# Autodesk Inventor assembly: Assembly_carcasa
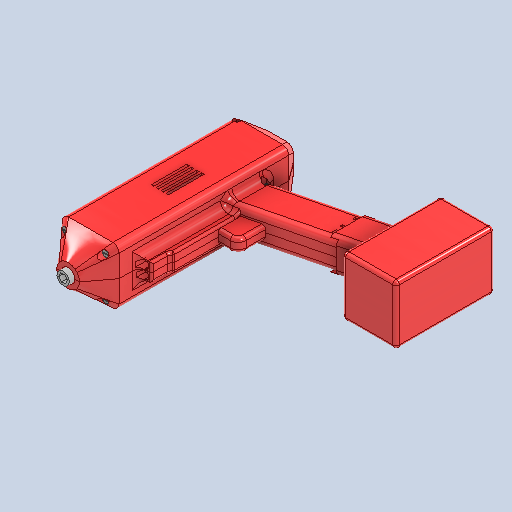
[picture p0: Inventor's stored thumbnail of the model, 512x512]
Saved by Autodesk Inventor 2025.2 (Build 292293000, 293)
## iProperties
Created: 2024-04-15
Part Number: Assembly_carcasa
Document SubType Name: Assembly
Designer: mirun
Author: mirun
## Documents named in this file (17)
- C:\Users\mirewn\Documents\GitHub\Electric-Screwdriver\Assembly.iam
- C:\Users\mirewn\Documents\Inventor\Content Center Files\R2025\en-US\DIN 439-2\DIN 439 - M3 x 0.5.ipt
- C:\Users\mirewn\Documents\Inventor\Content Center Files\R2025\en-US\DIN 934\DIN 934 - M3 x 0.5.ipt
- C:\Users\mirewn\Documents\Inventor\Content Center Files\R2025\en-US\DIN 963\DIN 963 - M3 x 16.ipt
- C:\Users\mirewn\Documents\Inventor\Content Center Files\R2025\en-US\DIN 912\DIN 912 - M3 x 0.5 x 12 x 10.75.ipt
- C:\Users\mirewn\Documents\Inventor\Content Center Files\R2025\en-US\DIN 912\DIN 912 - M3 x 0.5 x 30 x 18.ipt
- C:\Users\mirewn\Documents\Inventor\Content Center Files\R2025\en-US\DIN 912\DIN 912 - M3 x 0.5 x 20 x 18.75.ipt
- C:\Users\mirewn\Documents\Inventor\Content Center Files\R2025\en-US\DIN 912\DIN 912 - M3 x 0.5 x 16 x 14.75.ipt
- C:\Users\mirewn\Documents\GitHub\Electric-Screwdriver\battery_pack_lid.ipt
- C:\Users\mirewn\Documents\GitHub\Electric-Screwdriver\case_R.ipt
- C:\Users\mirewn\Documents\GitHub\Electric-Screwdriver\button.ipt
- C:\Users\mirewn\Documents\GitHub\Electric-Screwdriver\bit_adaptor.ipt
- C:\Users\mirewn\Documents\GitHub\Electric-Screwdriver\bit_adaptor_lid.ipt
- C:\Users\mirewn\Documents\GitHub\Electric-Screwdriver\case_L.ipt
- C:\Users\mirewn\Documents\GitHub\Electric-Screwdriver\GearBox\Assembly.iam
- C:\Users\mirewn\Documents\GitHub\Electric-Screwdriver\battery.ipt
- C:\Users\mirewn\Documents\GitHub\Electric-Screwdriver\battery_pack.ipt
## Components (32 placed, 16 different names)
1. case_R:1 — Mate:3, Mate:4, Flush:2, Mate:12, Mate:13, Flush:3, Flush:4, Mate:30, Mate:31, Mate:32, Mate:36, Mate:37, Mate:45, Mate:46, Mate:49, Mate:50, Mate:52, Mate:55, Insert:13, Insert:14
2. button:1 — Mate:3, Mate:4, Flush:2, Mate:45, Mate:46
3. bit_adaptor:1 — Mate:8, Mate:9, Mate:10, Mate:12, Mate:33
4. bit_adaptor_lid:1 — Mate:8, Mate:9, Mate:10
5. case_L:1 — Mate:13, Flush:3, Flush:4, Mate:35, Mate:47, Mate:48, Mate:51, Mate:53, Mate:54, Insert:15
6. DIN 934 - replaced by DIN EN 24032/28673/28674 M3:1 — Mate:53, Mate:54
7. DIN 934 - replaced by DIN EN 24032/28673/28674 M3:2 — Mate:51
8. DIN 934 - replaced by DIN EN 24032/28673/28674 M3:3 — Mate:52, Mate:55
9. Assembly:1 [sub-assembly] — Mate:30, Mate:31, Mate:32, Mate:33, Insert:1, Insert:2, Insert:3, Insert:4, Insert:5, Insert:6, Insert:7, Insert:8, Insert:9, Insert:10, Insert:11, Insert:12
10. battery:1 — Flush:5, Flush:6, Mate:34, Mate:42, Mate:43, Mate:44
11. battery:2 — Flush:5, Flush:6, Mate:34
12. battery_pack:1 — Mate:35, Mate:36, Mate:37, Mate:39, Mate:40, Mate:41, Mate:42, Mate:43, Mate:44
13. battery_pack_lid:1 — Mate:39, Mate:40, Mate:41
14. DIN 963 - replaced by DIN EN ISO 2009 M3 x 16:1 — Mate:47
15. DIN 963 - replaced by DIN EN ISO 2009 M3 x 16:2 — Mate:48
16. DIN 963 - replaced by DIN EN ISO 2009 M3 x 16:3 — Mate:49
17. DIN 963 - replaced by DIN EN ISO 2009 M3 x 16:4 — Mate:50
18. DIN 439-2 - replaced by DIN EN 24035/28675 M3:1 — Insert:1
19. DIN 439-2 - replaced by DIN EN 24035/28675 M3:2 — Insert:2
20. DIN 439-2 - replaced by DIN EN 24035/28675 M3:3 — Insert:3
21. DIN 439-2 - replaced by DIN EN 24035/28675 M3:4 — Insert:4
22. DIN 912 - replaced by DIN EN ISO 4762 M3 x 12:1 — Insert:5
23. DIN 912 - replaced by DIN EN ISO 4762 M3 x 12:2 — Insert:6
24. DIN 912 - replaced by DIN EN ISO 4762 M3 x 12:3 — Insert:7
25. DIN 912 - replaced by DIN EN ISO 4762 M3 x 12:4 — Insert:8
26. DIN 439-2 - replaced by DIN EN 24035/28675 M3:5 — Insert:9
27. DIN 439-2 - replaced by DIN EN 24035/28675 M3:6 — Insert:10
28. DIN 439-2 - replaced by DIN EN 24035/28675 M3:7 — Insert:11
29. DIN 439-2 - replaced by DIN EN 24035/28675 M3:8 — Insert:12
30. DIN 912 - replaced by DIN EN ISO 4762 M3 x 30:1 — Insert:13
31. DIN 912 - replaced by DIN EN ISO 4762 M3 x 20:1 — Insert:14
32. DIN 912 - replaced by DIN EN ISO 4762 M3 x 16:1 — Insert:15
## Relationships (56: Mate 36, Insert 15, Flush 5)
- Mate:3 (0.25 mm): case_R:1 ↔ button:1
- Mate:4: case_R:1 ↔ button:1
- Flush:2: case_R:1 ↔ button:1
- Mate:8: bit_adaptor:1 ↔ bit_adaptor_lid:1
- Mate:9: bit_adaptor:1 ↔ bit_adaptor_lid:1
- Mate:10: bit_adaptor:1 ↔ bit_adaptor_lid:1
- Mate:12: case_R:1 ↔ bit_adaptor:1
- Mate:13: case_R:1 ↔ case_L:1
- Flush:3: case_R:1 ↔ case_L:1
- Flush:4: case_R:1 ↔ case_L:1
- [Mate]: case_L:1 ↔ DIN 934 - replaced by DIN EN 24032/28673/28674 M3:1
- [Mate]: case_L:1 ↔ DIN 934 - replaced by DIN EN 24032/28673/28674 M3:2
- [Mate]: case_L:1 ↔ DIN 934 - replaced by DIN EN 24032/28673/28674 M3:2
- [Mate]: case_R:1 ↔ DIN 934 - replaced by DIN EN 24032/28673/28674 M3:3
- Mate:30: case_R:1 ↔ Assembly:1
- Mate:31: case_R:1 ↔ Assembly:1
- Mate:32 (1.5 mm): case_R:1 ↔ Assembly:1
- Mate:33: bit_adaptor:1 ↔ Assembly:1
- Flush:5: battery:1 ↔ battery:2
- Flush:6: battery:1 ↔ battery:2
- Mate:34 (2 mm): battery:1 ↔ battery:2
- Mate:35: case_L:1 ↔ battery_pack:1
- Mate:36 (0.25 mm): case_R:1 ↔ battery_pack:1
- Mate:37: case_R:1 ↔ battery_pack:1
- Mate:39: battery_pack:1 ↔ battery_pack_lid:1
- Mate:40: battery_pack:1 ↔ battery_pack_lid:1
- Mate:41: battery_pack:1 ↔ battery_pack_lid:1
- Mate:42 (1 mm): battery:1 ↔ battery_pack:1
- Mate:43 (1 mm): battery:1 ↔ battery_pack:1
- Mate:44 (1 mm): battery:1 ↔ battery_pack:1
- Mate:45: case_R:1 ↔ button:1
- Mate:46: case_R:1 ↔ button:1
- Mate:47: case_L:1 ↔ DIN 963 - replaced by DIN EN ISO 2009 M3 x 16:1
- Mate:48: case_L:1 ↔ DIN 963 - replaced by DIN EN ISO 2009 M3 x 16:2
- Mate:49: case_R:1 ↔ DIN 963 - replaced by DIN EN ISO 2009 M3 x 16:3
- Mate:50: case_R:1 ↔ DIN 963 - replaced by DIN EN ISO 2009 M3 x 16:4
- Insert:1: Assembly:1 ↔ DIN 439-2 - replaced by DIN EN 24035/28675 M3:1
- Insert:2: Assembly:1 ↔ DIN 439-2 - replaced by DIN EN 24035/28675 M3:2
- Insert:3: Assembly:1 ↔ DIN 439-2 - replaced by DIN EN 24035/28675 M3:3
- Insert:4: Assembly:1 ↔ DIN 439-2 - replaced by DIN EN 24035/28675 M3:4
- Insert:5: Assembly:1 ↔ DIN 912 - replaced by DIN EN ISO 4762 M3 x 12:1
- Insert:6: Assembly:1 ↔ DIN 912 - replaced by DIN EN ISO 4762 M3 x 12:2
- Insert:7: Assembly:1 ↔ DIN 912 - replaced by DIN EN ISO 4762 M3 x 12:3
- Insert:8: Assembly:1 ↔ DIN 912 - replaced by DIN EN ISO 4762 M3 x 12:4
- Insert:9: Assembly:1 ↔ DIN 439-2 - replaced by DIN EN 24035/28675 M3:5
- Insert:10: Assembly:1 ↔ DIN 439-2 - replaced by DIN EN 24035/28675 M3:6
- Insert:11: Assembly:1 ↔ DIN 439-2 - replaced by DIN EN 24035/28675 M3:7
- Insert:12: Assembly:1 ↔ DIN 439-2 - replaced by DIN EN 24035/28675 M3:8
- Mate:51: case_L:1 ↔ DIN 934 - replaced by DIN EN 24032/28673/28674 M3:2
- Mate:52: case_R:1 ↔ DIN 934 - replaced by DIN EN 24032/28673/28674 M3:3
- Mate:53: case_L:1 ↔ DIN 934 - replaced by DIN EN 24032/28673/28674 M3:1
- Mate:54 (0.15 mm): case_L:1 ↔ DIN 934 - replaced by DIN EN 24032/28673/28674 M3:1
- Mate:55 (0.625 mm): case_R:1 ↔ DIN 934 - replaced by DIN EN 24032/28673/28674 M3:3
- Insert:13: case_R:1 ↔ DIN 912 - replaced by DIN EN ISO 4762 M3 x 30:1
- Insert:14: case_R:1 ↔ DIN 912 - replaced by DIN EN ISO 4762 M3 x 20:1
- Insert:15: case_L:1 ↔ DIN 912 - replaced by DIN EN ISO 4762 M3 x 16:1
